# Autodesk Inventor assembly: Objective
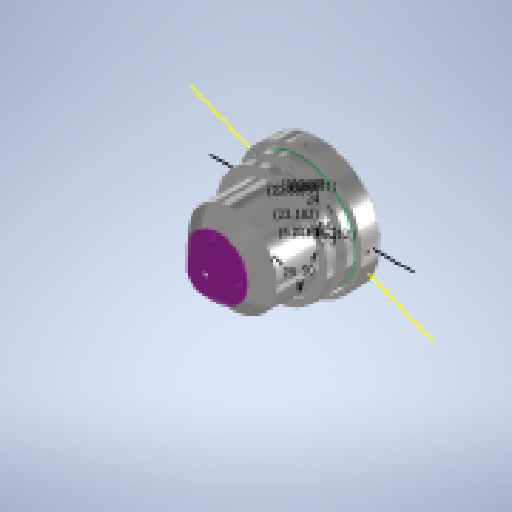
[picture p0: Inventor's stored thumbnail of the model, 512x512]
Saved by Autodesk Inventor 2023 (Build 270158000, 158)
## iProperties
Created: 2022-03-30
Part Number: Objective
Document SubType Name: Assembly
Designer: Vinicius Miguel
Author: Vinicius Miguel
## Documents named in this file (12)
- P:\SEM-Mechanical\Objective.iam
- P:\SEM-Mechanical\001.ipt
- P:\SEM-Mechanical\002.ipt
- P:\SEM-Mechanical\003.ipt
- P:\SEM-Mechanical\004.ipt
- P:\SEM-Mechanical\005.ipt
- P:\SEM-Mechanical\006.ipt
- P:\SEM-Mechanical\007.ipt
- P:\SEM-Mechanical\035.ipt
- P:\SEM-Mechanical\036.ipt
- P:\SEM-Mechanical\037.ipt
- P:\SEM-Mechanical\ScanningCoils.iam
## Components (11 placed, 11 different names)
1. 001:1 — Mate:1, Flush:1, Flush:2, Mate:3
2. 002:1 — Rotational:1, Rotational:2, Rotational:3
3. 003:1 — Mate:2, Mate:3, Flush:3, Mate:8
4. 004:1 — Rotational:2
5. 005:1 — Mate:7, Mate:8, Mate:10, Rotational:1, Mate:13, Rotational:6
6. 006:1 — Mate:9, Mate:10, Mate:11, Flush:4, Mate:13, Angle:1
7. 007:1 — Mate:11, Rotational:5, Mate:12
8. 035:1 — Rotational:3, Rotational:4
9. 036:1 — Rotational:4
10. 037:1 — Rotational:5, Mate:12
11. ScanningCoils:1 [sub-assembly] — Rotational:6, Angle:1
## Relationships (21: Mate 10, RevoluteJoint 6, Flush 4, Angle 1)
- Mate:1: 001:1
- Flush:1: 001:1
- Flush:2: 001:1
- Mate:2: 003:1
- Mate:3: 001:1 ↔ 003:1
- Flush:3: 003:1
- Mate:7: 005:1
- Mate:8: 003:1 ↔ 005:1
- Mate:9: 006:1
- Mate:10: 005:1 ↔ 006:1
- Mate:11: 006:1 ↔ 007:1
- Flush:4: 006:1
- Rotational:1 [RevoluteJoint]: 002:1 ↔ 005:1
- Rotational:2 [RevoluteJoint]: 002:1 ↔ 004:1
- Rotational:3 [RevoluteJoint]: 002:1 ↔ 035:1
- Rotational:4 [RevoluteJoint]: 035:1 ↔ 036:1
- Rotational:5 [RevoluteJoint]: 007:1 ↔ 037:1
- Mate:12: 007:1 ↔ 037:1
- Mate:13: 005:1 ↔ 006:1
- Rotational:6 [RevoluteJoint]: 005:1 ↔ ScanningCoils:1
- Angle:1 (0 deg): 006:1 ↔ ScanningCoils:1
